# Autodesk Inventor assembly: top_base
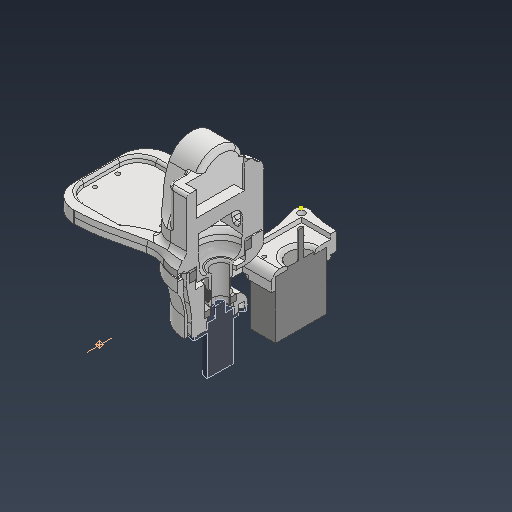
[picture p0: Inventor's stored thumbnail of the model, 512x512]
Saved by Autodesk Inventor 2026.1 (Build 301233020, 233B)
## iProperties
Created: 2025-12-12
Part Number: top_base
Document SubType Name: Assembly
Designer: Piter
Author: Piter
## Documents named in this file (7)
- C:\Users\Piter\OneDrive\Pulpit\Robots\david_Arm\Davie-Robot-Arm\3D Models\top_base.iam
- C:\Users\Piter\OneDrive\Pulpit\Robots\david_Arm\Davie-Robot-Arm\3D Models\Base_top.ipt
- C:\Users\Piter\OneDrive\Pulpit\Robots\david_Arm\Davie-Robot-Arm\3D Models\Component models\Slip_ring.ipt
- C:\Users\Piter\OneDrive\Pulpit\Robots\david_Arm\Davie-Robot-Arm\3D Models\Component models\small_bearing.ipt
- C:\Users\Piter\OneDrive\Pulpit\Robots\david_Arm\Davie-Robot-Arm\3D Models\Component models\big_bearing.ipt
- C:\Users\Piter\OneDrive\Pulpit\Robots\david_Arm\Davie-Robot-Arm\3D Models\Component models\Stepper.ipt
- C:\Users\Piter\OneDrive\Pulpit\Robots\david_Arm\Davie-Robot-Arm\3D Models\rotation_base_v3.ipt
## Components (6 placed, 6 different names)
1. Base_top:1 — Rigid:1, Rigid:2, Rotational:1, Rotational:2, Rotational:3
2. Slip_ring:1 — Rigid:1
3. small_bearing:1 — Rigid:2
4. big_bearing:1 — Rotational:1
5. Stepper:1 — Rotational:2
6. rotation_base_v3:1 — Rotational:3
## Relationships (5: RevoluteJoint 3, WeldJoint 2)
- Rigid:1 [WeldJoint]: Base_top:1 ↔ Slip_ring:1
- Rigid:2 [WeldJoint]: Base_top:1 ↔ small_bearing:1
- Rotational:1 [RevoluteJoint]: Base_top:1 ↔ big_bearing:1
- Rotational:2 [RevoluteJoint]: Base_top:1 ↔ Stepper:1
- Rotational:3 [RevoluteJoint] (-1 mm): Base_top:1 ↔ rotation_base_v3:1
